# Autodesk Inventor assembly: EnsamblajePalanca
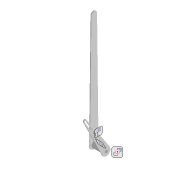
[picture p0: Inventor's stored thumbnail of the model, 180x180]
Saved by Autodesk Inventor 2021 (Build 250183000, 183)
## iProperties
Created: 2021-05-09
Part Number: EnsamblajePalanca
Document SubType Name: Assembly
Designer: carlo
Author: carlo
## Documents named in this file (4)
- C:\Users\carlo\Desktop\Planos\EnsamblajePalanca.iam
- C:\Users\carlo\Desktop\Planos\BrazoPalanca.ipt
- C:\Users\carlo\Desktop\Planos\CorrederaPalanca.ipt
- C:\Users\carlo\Desktop\Planos\UnionPalanca.ipt
## Components (3 placed, 3 different names)
1. BrazoPalanca:1 — Coincidencia:1, Coincidencia:2, Ángulo:1
2. CorrederaPalanca:1 — Coincidencia:3, Coincidencia:4, Ángulo:1
3. UnionPalanca:1 — Coincidencia:1, Coincidencia:2, Coincidencia:3, Coincidencia:4
## Relationships (5: Mate 4, Angle 1)
- Coincidencia:1 [Mate]: BrazoPalanca:1 ↔ UnionPalanca:1
- Coincidencia:2 [Mate]: BrazoPalanca:1 ↔ UnionPalanca:1
- Coincidencia:3 [Mate]: CorrederaPalanca:1 ↔ UnionPalanca:1
- Coincidencia:4 [Mate]: CorrederaPalanca:1 ↔ UnionPalanca:1
- Ángulo:1 [Angle] (26.9 deg): BrazoPalanca:1 ↔ CorrederaPalanca:1
